# Autodesk Inventor assembly: motor assembly_v2_MIR
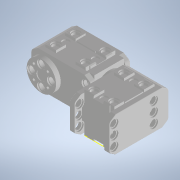
[picture p0: Inventor's stored thumbnail of the model, 180x180]
Saved by Autodesk Inventor 2021 (Build 250183000, 183)
## iProperties
Created: 2020-11-15
Part Number: motor assembly_v2_MIR
Document SubType Name: Assembly
Designer: Paco
Mass: 33.6452 g
Surface Area: 122.581 cm^2
Volume: 33.6452 cm^3
Density: 1 g/cm^3
Author: Paco
## Documents named in this file (3)
- E:\EPFL_MASTER\Sem proj\IISRD_CAD\final plane\motor assembly_v2_MIR.iam
- E:\EPFL_MASTER\Sem proj\IISRD_CAD\XL320XL-320_MIR.ipt
- E:\EPFL_MASTER\Sem proj\IISRD_CAD\final plane\XL_XL_interface_v2_MIR.ipt
## Components (3 placed, 2 different names)
1. XL320XL-320_MIR:1 — Mate:6, Mate:5, Mate:4
2. XL320XL-320_MIR:2 — Mate:2, Rotational:1
3. XL_XL_interface_v2_MIR:1 — Mate:6, Mate:5, Mate:4, Mate:2, Rotational:1
## Relationships (5: Mate 4, RevoluteJoint 1)
- Mate:6: XL320XL-320_MIR:1 ↔ XL_XL_interface_v2_MIR:1
- Mate:5: XL320XL-320_MIR:1 ↔ XL_XL_interface_v2_MIR:1
- Mate:4: XL320XL-320_MIR:1 ↔ XL_XL_interface_v2_MIR:1
- Mate:2: XL320XL-320_MIR:2 ↔ XL_XL_interface_v2_MIR:1
- Rotational:1 [RevoluteJoint]: XL320XL-320_MIR:2 ↔ XL_XL_interface_v2_MIR:1
